# Autodesk Inventor assembly: Handle Assembly
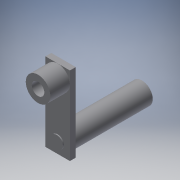
[picture p0: Inventor's stored thumbnail of the model, 180x180]
Saved by Autodesk Inventor 2018 (Build 220112000, 112)
## iProperties
Created: 2017-04-14
Part Number: Handle Assembly
Document SubType Name: Assembly
Designer: Administrator
Author: Administrator
## Documents named in this file (4)
- C:\Users\Administrator\Documents\TA202\Handle Assembly.iam
- C:\Users\Administrator\Documents\TA202\Handle Connected.ipt
- C:\Users\Administrator\Documents\TA202\Handle Fix.ipt
- C:\Users\Administrator\Documents\TA202\Handle Holder.ipt
## Components (3 placed, 3 different names)
1. Handle Connected:1 — Mate:1, Tangent:1, Tangent:2, Insert:1
2. Handle Fix:1 — Mate:1, Tangent:1, Tangent:2
3. Handle Holder:1 — Insert:1
## Relationships (4: Tangent 2, Mate 1, Insert 1)
- Mate:1: Handle Connected:1 ↔ Handle Fix:1
- Tangent:1: Handle Connected:1 ↔ Handle Fix:1
- Tangent:2: Handle Connected:1 ↔ Handle Fix:1
- Insert:1: Handle Connected:1 ↔ Handle Holder:1
